# Autodesk Inventor assembly: assembled-antenna
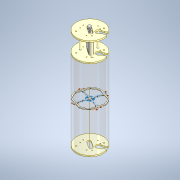
[picture p0: Inventor's stored thumbnail of the model, 180x180]
Saved by Autodesk Inventor 2021 (Build 250183000, 183)
## iProperties
Created: 2020-09-03
Part Number: assembled-antenna
Document SubType Name: Assembly
Designer: dsouthall
Author: dsouthall
## iProperties of the stored document inice_bottom.ipt
Created: 2020-11-16
Part Number: inice_bottom
Material: Generic
Document SubType Name: Modeling
Designer: dsouthall
Density: 1 g/cm^3
Appearance: Default
Author: dsouthall
Revision Number: ANY
## iProperties of the stored document inice_top.ipt
Created: 2020-11-16
Part Number: inice_top
Material: Generic
Document SubType Name: Modeling
Designer: dsouthall
Density: 1 g/cm^3
Appearance: Default
Author: dsouthall
Revision Number: ANY
## iProperties of the stored document front_end_box.iam
Created: 2020-11-16
Part Number: front_end_box
Description: STEP AP203
Document SubType Name: Assembly
Designer: dsouthall
Sending System: SolidWorks 2014
Preprocessor: SwSTEP 2.0
Title: front_end_box.STEP
Revision Number: ANY
## iProperties of the stored document fake_sma_with_cable.ipt
Created: 2020-11-16
Part Number: fake_sma_with_cable
Material: Generic
Document SubType Name: Modeling
Designer: dsouthall
Density: 1 g/cm^3
Appearance: Default
Author: dsouthall
Revision Number: ANY
## Documents named in this file (14)
- C:\Users\dsouthall\OneDrive - The University of Chicago\Hpol\hpol-prototype\design\Quad-Slot\Model 8 in\assembled-closed-antenna.iam
- C:\Users\dsouthall\OneDrive - The University of Chicago\Hpol\hpol-prototype\design\Quad-Slot\Model 8 in\assembled-feed.iam
- C:\Users\dsouthall\OneDrive - The University of Chicago\Hpol\hpol-prototype\design\Quad-Slot\Model 8 in\source\92141A003_TYPE 18-8 STAINLESS STEEL FLAT WASHER\92141A003_TYPE 18-8 STAINLESS STEEL FLAT WASHER.ipt
- C:\Users\dsouthall\OneDrive - The University of Chicago\Hpol\hpol-prototype\design\Quad-Slot\Model 8 in\source\96877A118_18-8 SS 82 DEG FLAT HEAD PHIL MACHINE SCREW\96877A118_18-8 SS 82 DEG FLAT HEAD PHIL MACHINE SCREW.ipt
- C:\Users\dsouthall\OneDrive - The University of Chicago\Hpol\hpol-prototype\design\Quad-Slot\Model 8 in\source\91841A003_TYPE 18-8 STAINLESS STEEL HEX NUT\91841A003_TYPE 18-8 STAINLESS STEEL HEX NUT.ipt
- C:\Users\dsouthall\OneDrive - The University of Chicago\Hpol\hpol-prototype\design\Quad-Slot\Model 8 in\source\my_faceplate.ipt
- C:\Users\dsouthall\OneDrive - The University of Chicago\Hpol\hpol-prototype\design\Quad-Slot\Model 8 in\source\my can\can_closed.ipt
- C:\Users\dsouthall\OneDrive - The University of Chicago\Hpol\hpol-prototype\design\Quad-Slot\Model 8 in\source\End Cap.ipt
- C:\Users\dsouthall\OneDrive - The University of Chicago\Hpol\hpol-prototype\design\Quad-Slot\Model 8 in\source\Short Support.ipt
- **C:\Users\dsouthall\OneDrive - The University of Chicago\Hpol\hpol-prototype\design\Quad-Slot\Model 8 in\assembled-closed-antenna.iam*LocalDocs*xAaaaamdaAaaaaaaaAaaaaxhxFa*front_end_box.iam
- **C:\Users\dsouthall\OneDrive - The University of Chicago\Hpol\hpol-prototype\design\Quad-Slot\Model 8 in\assembled-closed-antenna.iam*LocalDocs*xAaaaamaaAaaaaaaaAaaaq5zb4b*inice_bottom.ipt
- **C:\Users\dsouthall\OneDrive - The University of Chicago\Hpol\hpol-prototype\design\Quad-Slot\Model 8 in\assembled-closed-antenna.iam*LocalDocs*xAaaaacaaAaaaaaaaAaaaqa3yKc*inice_top.ipt
- **C:\Users\dsouthall\OneDrive - The University of Chicago\Hpol\hpol-prototype\design\Quad-Slot\Model 8 in\assembled-closed-antenna.iam*LocalDocs*xAaaaq4aaAaaaaaaaAaaaqf0qEa*fake_sma_with_cable.ipt
- C:\Users\dsouthall\OneDrive - The University of Chicago\Hpol\hpol-prototype\design\Quad-Slot\Model 8 in\source\front_end_box.STEP
## Components (35 placed, 9 different names)
1. can_closed:1 — Insert:25, Insert:26, Insert:37, Insert:38, Mate:4, Mate:5, Flush:1, Angle:4, Angle:5, Insert:39, Insert:40, Angle:8
2. my_faceplate:1 — Insert:37, Angle:3
3. my_faceplate:2 — Insert:38, Angle:3
4. assembled-feed:1 [sub-assembly] — Mate:5, Flush:1, Angle:4, Angle:5
5. End Cap:1 — Angle:6, Insert:39
6. End Cap:2 — Angle:6, Insert:40, Insert:41, Insert:42, Insert:43, Angle:7, Mate:7, Angle:8
7. End Cap:3 — Insert:44, Mate:6, Angle:7, Mate:8
8. Short Support:1 — Insert:41, Insert:44
9. Short Support:2 — Insert:42, Mate:6
10. Short Support:3 — Insert:43
11. front_end_box:1 [sub-assembly] — Mate:7, Mate:8
12. 92141A003_TYPE 18-8 STAINLESS STEEL FLAT WASHER:12 — Insert:35, Insert:36
13. 91841A003_TYPE 18-8 STAINLESS STEEL HEX NUT:3 — Insert:36
14. 96877A118_18-8 SS 82 DEG FLAT HEAD PHIL MACHINE SCREW:3 — Insert:26, Insert:35
15. 92141A003_TYPE 18-8 STAINLESS STEEL FLAT WASHER:13
16. 91841A003_TYPE 18-8 STAINLESS STEEL HEX NUT:7
17. 96877A118_18-8 SS 82 DEG FLAT HEAD PHIL MACHINE SCREW:7
18. 92141A003_TYPE 18-8 STAINLESS STEEL FLAT WASHER:14
19. 91841A003_TYPE 18-8 STAINLESS STEEL HEX NUT:8
20. 96877A118_18-8 SS 82 DEG FLAT HEAD PHIL MACHINE SCREW:8
21. 92141A003_TYPE 18-8 STAINLESS STEEL FLAT WASHER:15
22. 91841A003_TYPE 18-8 STAINLESS STEEL HEX NUT:9
23. 96877A118_18-8 SS 82 DEG FLAT HEAD PHIL MACHINE SCREW:9
24. 92141A003_TYPE 18-8 STAINLESS STEEL FLAT WASHER:11 — Insert:33, Insert:34
25. 91841A003_TYPE 18-8 STAINLESS STEEL HEX NUT:4 — Insert:34
26. 96877A118_18-8 SS 82 DEG FLAT HEAD PHIL MACHINE SCREW:4 — Insert:25, Insert:33
27. 92141A003_TYPE 18-8 STAINLESS STEEL FLAT WASHER:16
28. 91841A003_TYPE 18-8 STAINLESS STEEL HEX NUT:10
29. 96877A118_18-8 SS 82 DEG FLAT HEAD PHIL MACHINE SCREW:10
30. 92141A003_TYPE 18-8 STAINLESS STEEL FLAT WASHER:17
31. 91841A003_TYPE 18-8 STAINLESS STEEL HEX NUT:11
32. 96877A118_18-8 SS 82 DEG FLAT HEAD PHIL MACHINE SCREW:11
33. 92141A003_TYPE 18-8 STAINLESS STEEL FLAT WASHER:18
34. 91841A003_TYPE 18-8 STAINLESS STEEL HEX NUT:12
35. 96877A118_18-8 SS 82 DEG FLAT HEAD PHIL MACHINE SCREW:12
## Component patterns: (4 elements, first: 92141A003_TYPE 18-8 STAINLESS STEEL FLAT WASHER:12 + 91841A003_TYPE 18-8 STAINLESS STEEL HEX NUT:3 + 96877A118_18-8 SS 82 DEG FLAT HEAD PHIL MACHINE SCREW:3), (4 elements, first: 92141A003_TYPE 18-8 STAINLESS STEEL FLAT WASHER:11 + 91841A003_TYPE 18-8 STAINLESS STEEL HEX NUT:4 + 96877A118_18-8 SS 82 DEG FLAT HEAD PHIL MACHINE SCREW:4)
## Relationships (26: Insert 14, Angle 6, Mate 5, Flush 1)
- Insert:25: can_closed:1 ↔ 96877A118_18-8 SS 82 DEG FLAT HEAD PHIL MACHINE SCREW:4
- Insert:26: can_closed:1 ↔ 96877A118_18-8 SS 82 DEG FLAT HEAD PHIL MACHINE SCREW:3
- Insert:33 (-2.54 mm): 92141A003_TYPE 18-8 STAINLESS STEEL FLAT WASHER:11 ↔ 96877A118_18-8 SS 82 DEG FLAT HEAD PHIL MACHINE SCREW:4
- Insert:34: 92141A003_TYPE 18-8 STAINLESS STEEL FLAT WASHER:11 ↔ 91841A003_TYPE 18-8 STAINLESS STEEL HEX NUT:4
- Insert:35 (-2.54 mm): 92141A003_TYPE 18-8 STAINLESS STEEL FLAT WASHER:12 ↔ 96877A118_18-8 SS 82 DEG FLAT HEAD PHIL MACHINE SCREW:3
- Insert:36: 92141A003_TYPE 18-8 STAINLESS STEEL FLAT WASHER:12 ↔ 91841A003_TYPE 18-8 STAINLESS STEEL HEX NUT:3
- Insert:37: can_closed:1 ↔ my_faceplate:1
- Insert:38 (-9.652 mm): can_closed:1 ↔ my_faceplate:2
- Angle:3 (0 deg): my_faceplate:1 ↔ my_faceplate:2
- Mate:4 (600 mm): can_closed:1
- Mate:5: can_closed:1 ↔ assembled-feed:1
- Flush:1 (-299.2 mm): can_closed:1 ↔ assembled-feed:1
- Angle:4 (0 deg): can_closed:1 ↔ assembled-feed:1
- Angle:5 (0 deg): can_closed:1 ↔ assembled-feed:1
- Angle:6 (0 deg): End Cap:1 ↔ End Cap:2
- Insert:39 (0.174 mm): can_closed:1 ↔ End Cap:1
- Insert:40 (-9.826 mm): can_closed:1 ↔ End Cap:2
- Insert:41: End Cap:2 ↔ Short Support:1
- Insert:42: End Cap:2 ↔ Short Support:2
- Insert:43: End Cap:2 ↔ Short Support:3
- Insert:44: End Cap:3 ↔ Short Support:1
- Mate:6: End Cap:3 ↔ Short Support:2
- Angle:7 (0 deg): End Cap:2 ↔ End Cap:3
- Mate:7 (6.35 mm): End Cap:2 ↔ front_end_box:1
- Mate:8 (1 mm): End Cap:3 ↔ front_end_box:1
- Angle:8 (0 deg): can_closed:1 ↔ End Cap:2
